# Autodesk Inventor assembly: UTM_Assembly
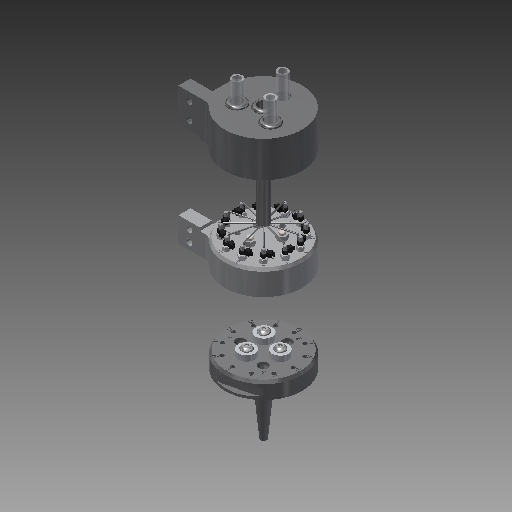
[picture p0: Inventor's stored thumbnail of the model, 512x512]
Saved by Autodesk Inventor 2017 (Build 210142000, 142)
## iProperties
Created: 2016-12-31
Part Number: UTM_Assembly
Document SubType Name: Assembly
Designer: umr
Author: umr
## Documents named in this file (13)
- D:\SeniorProject\Models2\UTM\UTM_Assembly.iam
- D:\SeniorProject\Models2\UTM\UTM Cover.ipt
- D:\SeniorProject\Models2\UTM\UTM.ipt
- D:\SeniorProject\Models2\UTM\12 wire cable.ipt
- D:\SeniorProject\Models2\UTM\1.5mm Square O-Ring 7.5mm ID (modelled as 8mm ID).ipt
- D:\SeniorProject\Models2\UTM\Grommet 9600k33.ipt
- D:\SeniorProject\Models2\UTM\Tubing.ipt
- D:\SeniorProject\Models2\UTM\M3 Screw_30mm.ipt
- D:\SeniorProject\Models2\UTM\M3 Spring 94125K472.ipt
- D:\SeniorProject\Models2\UTM\M3 Locknut.ipt
- D:\SeniorProject\Models2\UTM\Zip Tie.ipt
- D:\SeniorProject\Models2\UTM\MagnetAssembly.iam
- D:\SeniorProject\Models2\HeadTools\Seeder\SeederAssembly.iam
## Components (54 placed, 12 different names)
1. UTM Cover:1 — Mate:1, Flush:1, Mate:2, Mate:6, Mate:7, Mate:8, Mate:30, Mate:31, Mate:32, Mate:33, Mate:34, Flush:2, Flush:3, Flush:4
2. UTM:1 — Mate:1, Flush:1, Mate:3, Mate:4, Mate:5, Mate:13, Mate:16, Mate:19, Mate:22, Mate:23, Mate:24, Mate:25, Mate:26, Mate:27, Mate:28, Mate:34
3. 12 wire cable:1 — Mate:2, Mate:9
4. 1.5mm Square O-Ring 7.5mm ID (modelled as 8mm ID):1 — Mate:5
5. 1.5mm Square O-Ring 7.5mm ID (modelled as 8mm ID):2 — Mate:4
6. 1.5mm Square O-Ring 7.5mm ID (modelled as 8mm ID):3 — Mate:3
7. Grommet 9600k33:1 — Mate:9, Mate:31
8. Grommet 9600k33:2 — Mate:10, Mate:33
9. Grommet 9600k33:3 — Mate:12, Mate:32
10. Grommet 9600k33:4 — Mate:11, Mate:30
11. Tubing:1 — Mate:8, Mate:12, Flush:2
12. Tubing:2 — Mate:7, Mate:11, Flush:4
13. Tubing:3 — Mate:6, Mate:10, Flush:3
14. M3 Spring 94125K472:1 — Mate:15, Mate:16, Mate:17
15. MagnetAssembly:1 [sub-assembly] — Mate:22, Mate:27
16. MagnetAssembly:2 [sub-assembly] — Mate:23, Mate:26, Mate:35
17. MagnetAssembly:3 [sub-assembly] — Mate:24, Mate:25
18. SeederAssembly:1 [sub-assembly] — Mate:28, Mate:35
19. M3 Screw_30mm:1 — Mate:13, Mate:15, Mate:17, Mate:18, Mate:20
20. Zip Tie:1 — Mate:20, Mate:21
21. M3 Locknut:1 — Mate:18, Mate:19, Mate:21
22. M3 Screw_30mm:2
23. Zip Tie:2
24. M3 Locknut:2
25. M3 Screw_30mm:3
26. Zip Tie:3
27. M3 Locknut:3
28. M3 Screw_30mm:4
29. Zip Tie:4
30. M3 Locknut:4
31. M3 Screw_30mm:5
32. Zip Tie:5
33. M3 Locknut:5
34. M3 Screw_30mm:6
35. Zip Tie:6
36. M3 Locknut:6
37. M3 Screw_30mm:7
38. Zip Tie:7
39. M3 Locknut:7
40. M3 Screw_30mm:8
41. Zip Tie:8
42. M3 Locknut:8
43. M3 Screw_30mm:9
44. Zip Tie:9
45. M3 Locknut:9
46. M3 Screw_30mm:10
47. Zip Tie:10
48. M3 Locknut:10
49. M3 Screw_30mm:11
50. Zip Tie:11
51. M3 Locknut:11
52. M3 Screw_30mm:12
53. Zip Tie:12
54. M3 Locknut:12
## Component patterns: (12 elements, first: M3 Screw_30mm:1 + Zip Tie:1 + M3 Locknut:1)
## Relationships (37: Mate 33, Flush 4)
- Mate:1: UTM Cover:1 ↔ UTM:1
- Flush:1: UTM Cover:1 ↔ UTM:1
- Mate:2: UTM Cover:1 ↔ 12 wire cable:1
- Mate:3: UTM:1 ↔ 1.5mm Square O-Ring 7.5mm ID (modelled as 8mm ID):3
- Mate:4: UTM:1 ↔ 1.5mm Square O-Ring 7.5mm ID (modelled as 8mm ID):2
- Mate:5: UTM:1 ↔ 1.5mm Square O-Ring 7.5mm ID (modelled as 8mm ID):1
- Mate:6: UTM Cover:1 ↔ Tubing:3
- Mate:7: UTM Cover:1 ↔ Tubing:2
- Mate:8: UTM Cover:1 ↔ Tubing:1
- Mate:9: 12 wire cable:1 ↔ Grommet 9600k33:1
- Mate:10: Grommet 9600k33:2 ↔ Tubing:3
- Mate:11: Grommet 9600k33:4 ↔ Tubing:2
- Mate:12: Grommet 9600k33:3 ↔ Tubing:1
- Mate:13: UTM:1 ↔ M3 Screw_30mm:1
- Mate:15: M3 Spring 94125K472:1 ↔ M3 Screw_30mm:1
- Mate:16: UTM:1 ↔ M3 Spring 94125K472:1
- Mate:17: M3 Spring 94125K472:1 ↔ M3 Screw_30mm:1
- Mate:18: M3 Screw_30mm:1 ↔ M3 Locknut:1
- Mate:19: UTM:1 ↔ M3 Locknut:1
- Mate:20: M3 Screw_30mm:1 ↔ Zip Tie:1
- Mate:21: Zip Tie:1 ↔ M3 Locknut:1
- Mate:22: UTM:1 ↔ MagnetAssembly:1
- Mate:23: UTM:1 ↔ MagnetAssembly:2
- Mate:24: UTM:1 ↔ MagnetAssembly:3
- Mate:25: UTM:1 ↔ MagnetAssembly:3
- Mate:26: UTM:1 ↔ MagnetAssembly:2
- Mate:27: UTM:1 ↔ MagnetAssembly:1
- Mate:28: UTM:1 ↔ SeederAssembly:1
- Mate:30: UTM Cover:1 ↔ Grommet 9600k33:4
- Mate:31: UTM Cover:1 ↔ Grommet 9600k33:1
- Mate:32: UTM Cover:1 ↔ Grommet 9600k33:3
- Mate:33: UTM Cover:1 ↔ Grommet 9600k33:2
- Mate:34 (100 mm): UTM Cover:1 ↔ UTM:1
- Flush:2 (-20 mm): UTM Cover:1 ↔ Tubing:1
- Flush:3 (-20 mm): UTM Cover:1 ↔ Tubing:3
- Flush:4 (-20 mm): UTM Cover:1 ↔ Tubing:2
- Mate:35 (70 mm): MagnetAssembly:2 ↔ SeederAssembly:1
